# Autodesk Inventor assembly: Orangatang_Kegel
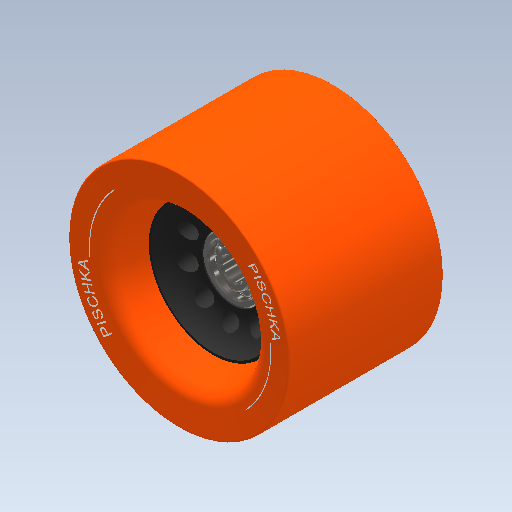
[picture p0: Inventor's stored thumbnail of the model, 512x512]
Saved by Autodesk Inventor 2020.1 (Build 241239000, 239)
## iProperties
Created: 2018-07-26
Part Number: Orangatang_Kegel
Document SubType Name: Assembly
Designer: Tobias
Mass: 277.486 g
Surface Area: 474.561 cm^2
Volume: 208.405 cm^3
Density: 1.33148 g/cm^3
Author: Tobias
## Documents named in this file (5)
- D:\OMG\E-Board\CAD\Inventor\Trucks\Orangatang Kegel\Orangatang_Kegel.iam
- D:\OMG\E-Board\CAD\Inventor\Trucks\Orangatang Kegel\Kegel_core.ipt
- D:\OMG\E-Board\CAD\Inventor\Trucks\Orangatang Kegel\Kegel_urethane.ipt
- D:\OMG\E-Board\CAD\Inventor\Trucks\spacer.ipt
- D:\OMG\E-Board\CAD\Inventor\Trucks\Bearings\bearing_abec7.iam
## Components (5 placed, 4 different names)
1. Kegel_core:1 — Mate:1, Flush:3, Flush:4, Mate:4, Mate:5, Mate:6, Insert:1, Insert:3
2. Kegel_urethane:1 — Mate:4, Mate:5, Mate:6
3. spacer:1 — Insert:2
4. bearing_abec7:1 [sub-assembly] — Insert:1, Insert:2
5. bearing_abec7:2 [sub-assembly] — Insert:3
## Relationships (9: Mate 4, Insert 3, Flush 2)
- Mate:1: Kegel_core:1
- Flush:3: Kegel_core:1
- Flush:4: Kegel_core:1
- Mate:4: Kegel_core:1 ↔ Kegel_urethane:1
- Mate:5: Kegel_core:1 ↔ Kegel_urethane:1
- Mate:6: Kegel_core:1 ↔ Kegel_urethane:1
- Insert:1: Kegel_core:1 ↔ bearing_abec7:1
- Insert:2: spacer:1 ↔ bearing_abec7:1
- Insert:3: Kegel_core:1 ↔ bearing_abec7:2
